# Autodesk Inventor assembly: правый привод
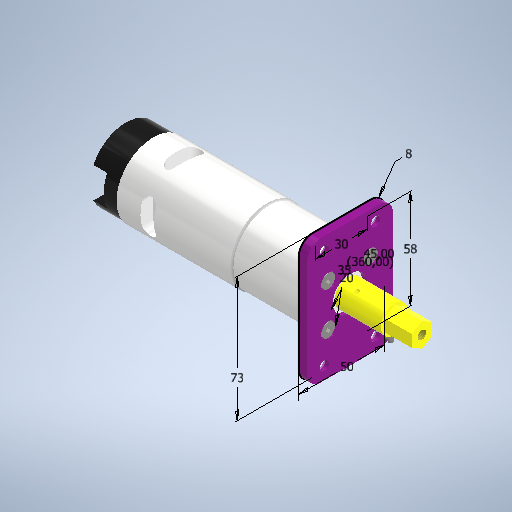
[picture p0: Inventor's stored thumbnail of the model, 512x512]
Saved by Autodesk Inventor 2025 (Build 290162000, 162)
## iProperties
Created: 2025-02-16
Part Number: правый привод
Document SubType Name: Assembly
Designer: volko
Author: volko
## Documents named in this file (7)
- C:\Users\volko\Desktop\диплом\Модели\детали\правый привод.iam
- C:\Users\volko\Desktop\диплом\Модели\Mecanum wheel - right\Mecanum wheel - right.iam
- C:\Users\volko\Desktop\диплом\Модели\детали\CHP-42GP-775 ABHL.ipt
- C:\Users\volko\Desktop\диплом\Модели\детали\кронштейн.ipt
- C:\Users\volko\Desktop\диплом\Модели\детали\переходная втулка.ipt
- C:\Users\volko\Desktop\диплом\Модели\детали\стандартные изделия\ru-RU\DIN 7991(2)\DIN 7991 - M4x8.ipt
- C:\Users\volko\Desktop\диплом\Модели\детали\стандартные изделия\ru-RU\DIN 913\DIN 913 - M3 x 5.ipt
## Components (9 placed, 6 different names)
1. Mecanum wheel - right:1 [sub-assembly] — Совмещение:8, Совмещение:9, Совмещение:10, Совмещение:12
2. CHP-42GP-775 ABHL:1 — Совмещение:1, Совмещение:2, Заподлицо:1, Совмещение:3, Совмещение:5, Совмещение:6, Совмещение:7, Совмещение:11
3. кронштейн:1 — Совмещение:3, Совмещение:5, Совмещение:11, Совмещение:13, Совмещение:14, Совмещение:15, Совмещение:16
4. переходная втулка:1 — Совмещение:6, Совмещение:7, Совмещение:8, Совмещение:9, Совмещение:10, Совмещение:17
5. DIN 913 M3 x 5:1 — Совмещение:17
6. DIN 7991 M4x8:4 — Совмещение:16
7. DIN 7991 M4x8:3 — Совмещение:15
8. DIN 7991 M4x8:2 — Совмещение:14
9. DIN 7991 M4x8:1 — Совмещение:13
## Relationships (17: Mate 16, Flush 1)
- Совмещение:1 [Mate]: CHP-42GP-775 ABHL:1
- Совмещение:2 [Mate]: CHP-42GP-775 ABHL:1
- Заподлицо:1 [Flush]: CHP-42GP-775 ABHL:1
- Совмещение:3 [Mate]: CHP-42GP-775 ABHL:1 ↔ кронштейн:1
- Совмещение:5 [Mate]: CHP-42GP-775 ABHL:1 ↔ кронштейн:1
- Совмещение:6 [Mate]: CHP-42GP-775 ABHL:1 ↔ переходная втулка:1
- Совмещение:7 [Mate]: CHP-42GP-775 ABHL:1 ↔ переходная втулка:1
- Совмещение:8 [Mate]: Mecanum wheel - right:1 ↔ переходная втулка:1
- Совмещение:9 [Mate]: Mecanum wheel - right:1 ↔ переходная втулка:1
- Совмещение:10 [Mate]: Mecanum wheel - right:1 ↔ переходная втулка:1
- Совмещение:11 [Mate]: CHP-42GP-775 ABHL:1 ↔ кронштейн:1
- Совмещение:12 [Mate]: Mecanum wheel - right:1
- Совмещение:13 [Mate]: кронштейн:1 ↔ DIN 7991 M4x8:1
- Совмещение:14 [Mate]: кронштейн:1 ↔ DIN 7991 M4x8:2
- Совмещение:15 [Mate]: кронштейн:1 ↔ DIN 7991 M4x8:3
- Совмещение:16 [Mate]: кронштейн:1 ↔ DIN 7991 M4x8:4
- Совмещение:17 [Mate]: переходная втулка:1 ↔ DIN 913 M3 x 5:1
